# Autodesk Inventor assembly: CompleteAssembly
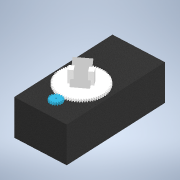
[picture p0: Inventor's stored thumbnail of the model, 180x180]
Saved by Autodesk Inventor 2022.2 (Build 262287010, 287A)
## iProperties
Created: 2022-05-02
Part Number: CompleteAssembly
Document SubType Name: Assembly
Designer: mabel
Author: mabel
## Documents named in this file (12)
- D:\GitHub\laser-nav\Mechanics\Final Prototype\CAD\CompleteAssembly.iam
- C:\Users\mabel\OneDrive\Documentos\Inventor\LaserNavigationSystem\TapaconEjeM.ipt
- C:\Users\mabel\OneDrive\Documentos\Inventor\LaserNavigationSystem\Cambio\EngraneN18.ipt
- C:\Users\mabel\OneDrive\Documentos\Inventor\LaserNavigationSystem\Cambio\EngraneN72.ipt
- C:\Users\mabel\OneDrive\Documentos\Inventor\LaserNavigationSystem\Mecanizado\Caja.ipt
- C:\Users\mabel\OneDrive\Documentos\Inventor\LaserNavigationSystem\Base.ipt
- C:\Users\mabel\OneDrive\Documentos\Inventor\LaserNavigationSystem\BaseL.ipt
- C:\Users\mabel\OneDrive\Documentos\Inventor\LaserNavigationSystem\BeamSplitter.ipt
- C:\Users\mabel\OneDrive\Documentos\Inventor\LaserNavigationSystem\Cambio\SoportaEspejo.ipt
- C:\Users\mabel\OneDrive\Documentos\Inventor\LaserNavigationSystem\Lente.ipt
- C:\Users\mabel\OneDrive\Documentos\Inventor\LaserNavigationSystem\SoporteLenteV2.ipt
- D:\GitHub\laser-nav\Mechanics\Final Prototype\CAD\SensorSupport.ipt
## Components (11 placed, 11 different names)
1. Gear-N18:1 — Coincidencia:3, Coincidencia:22
2. Gear-N72:1 — Coincidencia:1, Coincidencia:2, Coincidencia:23, Coincidencia:24, Coincidencia:25
3. Cover:1 — Coincidencia:1, Coincidencia:2, Coincidencia:3, Nivelación:1, Nivelación:2, Coincidencia:22
4. DarkBox:1 — Nivelación:1, Nivelación:2, Coincidencia:4, Coincidencia:5, Coincidencia:6, Coincidencia:7, Coincidencia:8, Coincidencia:9, Coincidencia:27, Coincidencia:29, Coincidencia:30
5. BaseBeamSplitterD:1 — Coincidencia:4, Coincidencia:5, Coincidencia:6, Coincidencia:12
6. BaseBeamSplitterL:1 — Coincidencia:7, Coincidencia:8, Coincidencia:9, Coincidencia:13
7. BeamSplitter:1 — Coincidencia:12, Coincidencia:13
8. MirrorSupport:1 — Coincidencia:23, Coincidencia:24, Coincidencia:25
9. Lens:1 — Coincidencia:28
10. LensSupport:1 — Coincidencia:27, Coincidencia:28
11. SensorSupport:1 — Coincidencia:29, Coincidencia:30
## Relationships (21: Mate 19, Flush 2)
- Coincidencia:1 [Mate]: Gear-N72:1 ↔ Cover:1
- Coincidencia:2 [Mate]: Gear-N72:1 ↔ Cover:1
- Coincidencia:3 [Mate]: Gear-N18:1 ↔ Cover:1
- Nivelación:1 [Flush]: Cover:1 ↔ DarkBox:1
- Nivelación:2 [Flush]: Cover:1 ↔ DarkBox:1
- Coincidencia:4 [Mate]: DarkBox:1 ↔ BaseBeamSplitterD:1
- Coincidencia:5 [Mate]: DarkBox:1 ↔ BaseBeamSplitterD:1
- Coincidencia:6 [Mate]: DarkBox:1 ↔ BaseBeamSplitterD:1
- Coincidencia:7 [Mate]: DarkBox:1 ↔ BaseBeamSplitterL:1
- Coincidencia:8 [Mate]: DarkBox:1 ↔ BaseBeamSplitterL:1
- Coincidencia:9 [Mate]: DarkBox:1 ↔ BaseBeamSplitterL:1
- Coincidencia:12 [Mate]: BaseBeamSplitterD:1 ↔ BeamSplitter:1
- Coincidencia:13 [Mate]: BaseBeamSplitterL:1 ↔ BeamSplitter:1
- Coincidencia:22 [Mate]: Gear-N18:1 ↔ Cover:1
- Coincidencia:23 [Mate]: Gear-N72:1 ↔ MirrorSupport:1
- Coincidencia:24 [Mate]: Gear-N72:1 ↔ MirrorSupport:1
- Coincidencia:25 [Mate]: Gear-N72:1 ↔ MirrorSupport:1
- Coincidencia:27 [Mate]: DarkBox:1 ↔ LensSupport:1
- Coincidencia:28 [Mate]: Lens:1 ↔ LensSupport:1
- Coincidencia:29 [Mate]: DarkBox:1 ↔ SensorSupport:1
- Coincidencia:30 [Mate]: DarkBox:1 ↔ SensorSupport:1
